# Autodesk Inventor assembly: NoStandAssem
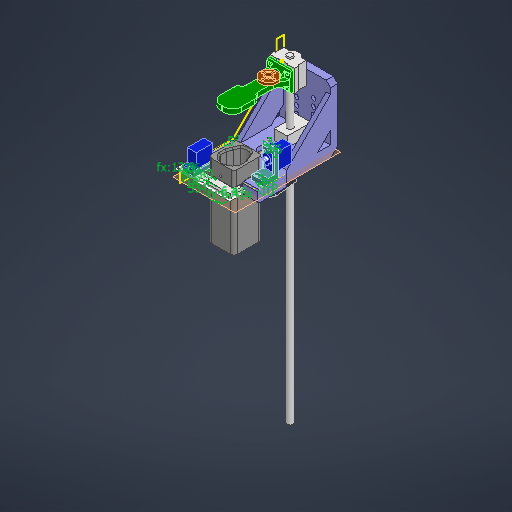
[picture p0: Inventor's stored thumbnail of the model, 512x512]
Saved by Autodesk Inventor 2025.1 (Build 291241000, 241)
## iProperties
Created: 2025-02-18
Part Number: NoStandAssem
Document SubType Name: Assembly
Designer: 13156
Author: 13156
## Documents named in this file (15)
- C:\Users\jerem\Documents\GitHub\Perovskite-Automated-Synthesis-System\CAD\Pipette\NoStandAssem.iam
- C:\Users\jerem\Documents\GitHub\Perovskite-Automated-Synthesis-System\CAD\Pipette\HolderWStepper.ipt
- C:\Users\jerem\Documents\GitHub\Perovskite-Automated-Synthesis-System\CAD\Pipette\SLEEVE.ipt
- C:\Users\jerem\Documents\GitHub\Perovskite-Automated-Synthesis-System\CAD\Pipette\ServoHolder.ipt
- C:\Users\jerem\Documents\GitHub\Perovskite-Automated-Synthesis-System\CAD\Pipette\ServoHolder - short.ipt
- C:\Users\jerem\Documents\GitHub\Perovskite-Automated-Synthesis-System\CAD\Non 3D Printed Parts\Motors and Servos\NEMA17 Stepper Motor - 26 mm.ipt
- C:\Users\jerem\Documents\GitHub\Perovskite-Automated-Synthesis-System\CAD\Non 3D Printed Parts\Motors and Servos\SG90 Servo.ipt
- C:\Users\jerem\Documents\GitHub\Perovskite-Automated-Synthesis-System\CAD\Non 3D Printed Parts\Linear Rails\Linear Rod Holder SK8.ipt
- C:\Users\jerem\Documents\GitHub\Perovskite-Automated-Synthesis-System\CAD\Non 3D Printed Parts\Linear Rails\Linear Bearing 8mm Square.ipt
- C:\Users\jerem\Documents\GitHub\Perovskite-Automated-Synthesis-System\CAD\Non 3D Printed Parts\Linear Rails\8mm Linear Rod.ipt
- C:\Users\jerem\Documents\GitHub\Perovskite-Automated-Synthesis-System\CAD\Pipette\GrabberArm.ipt
- C:\Users\jerem\Documents\GitHub\Perovskite-Automated-Synthesis-System\CAD\Pipette\Actuator.ipt
- C:\Users\jerem\Documents\GitHub\Perovskite-Automated-Synthesis-System\CAD\Non 3D Printed Parts\Leadscrew.ipt
- C:\Users\jerem\Documents\GitHub\Perovskite-Automated-Synthesis-System\CAD\Non 3D Printed Parts\Motors and Servos\MG90s Arm.ipt
- C:\Users\jerem\Documents\GitHub\Perovskite-Automated-Synthesis-System\CAD\Pipette\arm2.ipt
## Components (15 placed, 14 different names)
1. HolderWStepper:1 — Mate:1, Mate:2, Flush:1, Mate:3, Mate:4, Mate:5, Mate:6, Mate:7, Mate:9, Mate:10, Mate:15, Mate:16, Mate:18, Mate:22, Mate:23, Mate:31, Angle:1
2. SLEEVE:1 — Mate:3, Mate:4, Mate:5
3. ServoHolder:1 — Mate:6, Mate:7, Mate:11, Mate:12
4. ServoHolder - short:1 — Mate:9, Mate:10, Mate:13, Mate:27, Mate:28, Mate:31
5. NEMA17 Stepper Motor - 26 mm:1 — Mate:22, Mate:23
6. SG90 Servo:1 — Mate:11, Mate:12
7. SG90 Servo:4 — Mate:13, Mate:27, Mate:28, Mate:29, Mate:32, Mate:33
8. Linear Rod Holder SK8:1 — Mate:16, Mate:17, Mate:18
9. Linear Bearing 8mm Square:1 — Mate:19, Mate:20, Mate:21, Angle:1
10. 8mm Linear Rod:1 — Mate:15, Mate:17, Mate:19
11. GrabberArm:1 — Mate:29, Mate:34
12. Actuator:2 — Mate:20, Mate:21, Mate:25, Mate:26
13. Leadscrew:1 — Mate:25, Mate:26
14. MG90s Arm:1 — Mate:32, Mate:33, Mate:34, Mate:35, Mate:36
15. arm2:1 — Mate:35, Mate:36
## Relationships (34: Mate 32, Flush 1, Angle 1)
- Mate:1: HolderWStepper:1
- Mate:2: HolderWStepper:1
- Flush:1: HolderWStepper:1
- Mate:3: HolderWStepper:1 ↔ SLEEVE:1
- Mate:4: HolderWStepper:1 ↔ SLEEVE:1
- Mate:5: HolderWStepper:1 ↔ SLEEVE:1
- Mate:6: HolderWStepper:1 ↔ ServoHolder:1
- Mate:7: HolderWStepper:1 ↔ ServoHolder:1
- Mate:9: HolderWStepper:1 ↔ ServoHolder - short:1
- Mate:10: HolderWStepper:1 ↔ ServoHolder - short:1
- Mate:11: ServoHolder:1 ↔ SG90 Servo:1
- Mate:12: ServoHolder:1 ↔ SG90 Servo:1
- Mate:13: ServoHolder - short:1 ↔ SG90 Servo:4
- Mate:15: HolderWStepper:1 ↔ 8mm Linear Rod:1
- Mate:16: HolderWStepper:1 ↔ Linear Rod Holder SK8:1
- Mate:17: Linear Rod Holder SK8:1 ↔ 8mm Linear Rod:1
- Mate:18: HolderWStepper:1 ↔ Linear Rod Holder SK8:1
- Mate:19: Linear Bearing 8mm Square:1 ↔ 8mm Linear Rod:1
- Mate:20: Linear Bearing 8mm Square:1 ↔ Actuator:2
- Mate:21: Linear Bearing 8mm Square:1 ↔ Actuator:2
- Mate:22: HolderWStepper:1 ↔ NEMA17 Stepper Motor - 26 mm:1
- Mate:23: HolderWStepper:1 ↔ NEMA17 Stepper Motor - 26 mm:1
- Mate:25: Actuator:2 ↔ Leadscrew:1
- Mate:26: Actuator:2 ↔ Leadscrew:1
- Mate:27: ServoHolder - short:1 ↔ SG90 Servo:4
- Mate:28: ServoHolder - short:1 ↔ SG90 Servo:4
- Mate:29: SG90 Servo:4 ↔ GrabberArm:1
- Mate:31: HolderWStepper:1 ↔ ServoHolder - short:1
- Angle:1 (0 deg): HolderWStepper:1 ↔ Linear Bearing 8mm Square:1
- Mate:32: SG90 Servo:4 ↔ MG90s Arm:1
- Mate:33: SG90 Servo:4 ↔ MG90s Arm:1
- Mate:34: GrabberArm:1 ↔ MG90s Arm:1
- Mate:35: MG90s Arm:1 ↔ arm2:1
- Mate:36: MG90s Arm:1 ↔ arm2:1
